# Autodesk Inventor assembly: BoltandTee
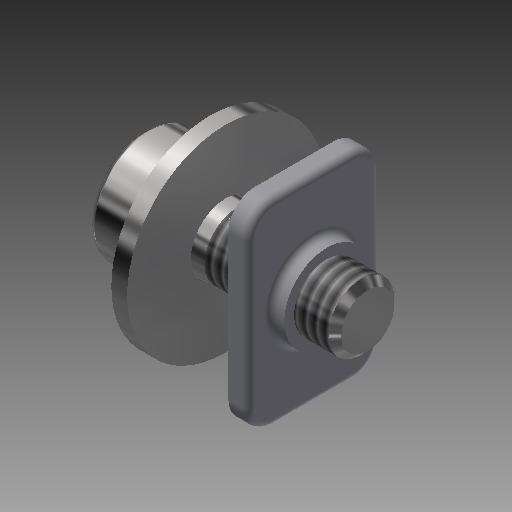
[picture p0: Inventor's stored thumbnail of the model, 512x512]
Saved by Autodesk Inventor 2018 (Build 220112000, 112)
## iProperties
Created: 2016-07-29
Part Number: BoltandTee
Document SubType Name: Assembly
Designer: User
Author: User
## Documents named in this file (4)
- C:\Users\Dan\OneDrive\SL-Inventor\The Beast v1.2 PackandGo\Workspaces\Workspace\BoltandTee.iam
- C:\Users\Dan\OneDrive\SL-Inventor\The Beast v1.2 PackandGo\Workspaces\Workspace\M5 Tee Nut-Generic_MIR_MIR.ipt
- C:\Users\Dan\OneDrive\SL-Inventor\The Beast v1.2 PackandGo\Workspaces\Workspace\en-US\ANSI B18.3.1M(6)\ANSI B18.3.1M - M5x0.8 x 12(1).ipt
- C:\Users\Dan\OneDrive\SL-Inventor\The Beast v1.2 PackandGo\Workspaces\Workspace\en-US\DIN 9021\DIN 9021 - 5.3.ipt
## Components (3 placed, 3 different names)
1. M5 Tee Nut-Generic_MIR_MIR:1
2. Forged Socket Head Cap Screw - Metric M5x0.8 x 12:1
3. DIN 9021 5.3:1
## Relationships (4: Mate 4)
- [Mate]: Forged Socket Head Cap Screw - Metric M5x0.8 x 12:1 ↔ DIN 9021 5.3:1
- [Mate]: Forged Socket Head Cap Screw - Metric M5x0.8 x 12:1 ↔ DIN 9021 5.3:1
- [Mate]: M5 Tee Nut-Generic_MIR_MIR:1 ↔ Forged Socket Head Cap Screw - Metric M5x0.8 x 12:1
- [Mate] (5.2 mm): M5 Tee Nut-Generic_MIR_MIR:1 ↔ DIN 9021 5.3:1
